# Autodesk Inventor assembly: 000-hand-grab-v5
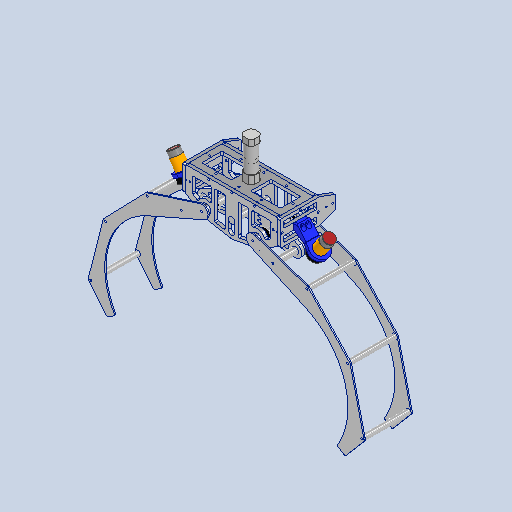
[picture p0: Inventor's stored thumbnail of the model, 512x512]
Saved by Autodesk Inventor 2025.2 (Build 292293000, 293)
## iProperties
Created: 2025-05-11
Part Number: 000-hand-grab-v5
Document SubType Name: Assembly
Designer: haruy
Author: haruy
## Documents named in this file (17)
- C:\Users\haruy\Documents\ロボコン\NHK2025\cad\nagahisa\hand\grab\000-hand-grab-v5.iam
- C:\Users\haruy\Documents\ロボコン\NHK2025\cad\nagahisa\hand\grab\hand-grab-v5-Plate-1.ipt
- C:\Users\haruy\Documents\ロボコン\NHK2025\cad\000_parts\エアシリンダー\airclinder\CDJ2B16-15Z-B(0_1_0).iam
- C:\Users\haruy\Documents\ロボコン\NHK2025\cad\nagahisa\hand\grab\hand-grab-v5-Plate-2.ipt
- C:\Users\haruy\Documents\ロボコン\NHK2025\cad\nagahisa\hand\grab\hand-grab-v5-Plate-3.ipt
- C:\Users\haruy\Documents\ロボコン\NHK2025\cad\000_parts\ベアリング\10\bear_10_15_sn.ipt
- C:\Users\haruy\Documents\ロボコン\NHK2025\cad\nagahisa\belt_liner\SCBRJ10-13.iam
- C:\Users\haruy\Documents\ロボコン\NHK2025\cad\nagahisa\hand\grab\hand-grab-v5-shaft-1.ipt
- C:\Users\haruy\Documents\ロボコン\NHK2025\cad\nagahisa\hand\grab\hand-grab-v5-Plate-4.ipt
- C:\Users\haruy\Documents\ロボコン\NHK2025\cad\nagahisa\hand\grab\hand-grab-v5-Plate-5.ipt
- C:\Users\haruy\Documents\ロボコン\NHK2025\cad\nagahisa\hand\grab\000-hand-grab-v5\デザイン アクセラレータ\平歯車1.iam
- C:\Users\haruy\Documents\ロボコン\NHK2025\cad\nagahisa\belt_liner\PSCTW10.iam
- C:\Users\haruy\Documents\ロボコン\NHK2025\cad\nagahisa\hand\grab\hand-grab-v5-shaft-2.ipt
- C:\Users\haruy\Documents\ロボコン\NHK2025\cad\nagahisa\hand\grab\hand-grab-v5-shaft-3.ipt
- C:\Users\haruy\Documents\ロボコン\NHK2025\cad\nagahisa\hand\grab\hand-grab-v5-3DP-1.ipt
- C:\Users\haruy\Documents\ロボコン\NHK2025\cad\000_parts\センサー\E18_D80NK.ipt
- C:\Users\haruy\Documents\ロボコン\NHK2025\cad\nagahisa\hand\grab\hand-grab-v5-shaft-4.ipt
## Components (38 placed, 16 different names)
1. hand-grab-v5-Plate-1:1 — 挿入:1, 角度:1, フラッシュ:7, メイト:3, メイト:4, フラッシュ:10, メイト:6, フラッシュ:12, メイト:8, フラッシュ:13
2. CDJ2B16-15Z-B(0_1_0):1 [sub-assembly] — 挿入:1, 挿入:2
3. hand-grab-v5-Plate-2:1 — 挿入:2, 角度:1, 挿入:27, フラッシュ:14
4. bear_10_15_sn:1 — 挿入:9, 挿入:22
5. bear_10_15_sn:2 — 挿入:10, 挿入:23
6. bear_10_15_sn:3 — 挿入:8, 挿入:21
7. bear_10_15_sn:4 — 挿入:7, 挿入:20
8. SCBRJ10-13:1 [sub-assembly] — 挿入:7, 挿入:46
9. SCBRJ10-13:2 [sub-assembly] — 挿入:8
10. SCBRJ10-13:3 [sub-assembly] — 挿入:9, 挿入:48
11. SCBRJ10-13:4 [sub-assembly] — 挿入:10
12. hand-grab-v5-shaft-1:1 — 挿入:15, 挿入:16, 挿入:25
13. hand-grab-v5-shaft-1:2 — 挿入:13, 挿入:14, 挿入:24
14. hand-grab-v5-Plate-4:1 — 挿入:13, 挿入:29, 挿入:32, 挿入:39, 挿入:51
15. hand-grab-v5-Plate-4:2 — 挿入:14, 挿入:28, 挿入:33, 挿入:38
16. hand-grab-v5-Plate-4:3 — 挿入:16, 挿入:30, 挿入:35, 挿入:37, 挿入:53
17. hand-grab-v5-Plate-4:4 — 挿入:15, 挿入:31, 挿入:34, 挿入:36
18. hand-grab-v5-Plate-5:1 — メイト:4, フラッシュ:10, メイト:7, 挿入:42, 挿入:43
19. hand-grab-v5-Plate-5:2 — フラッシュ:7, メイト:3, メイト:9, 挿入:40, 挿入:41
20. 平歯車:1 [sub-assembly] — 挿入:46, 挿入:47, 挿入:50
21. PSCTW10:1 [sub-assembly] — 挿入:47
22. 平歯車:2 [sub-assembly] — 挿入:48, 挿入:49, フラッシュ:14, 挿入:52
23. PSCTW10:2 [sub-assembly] — 挿入:49
24. hand-grab-v5-Plate-3:1 — メイト:6, フラッシュ:12, メイト:7, 挿入:20, 挿入:22, 挿入:24, 挿入:25
25. hand-grab-v5-Plate-3:2 — メイト:8, フラッシュ:13, メイト:9, 挿入:21, 挿入:23
26. hand-grab-v5-shaft-2:1 — 挿入:27
27. hand-grab-v5-shaft-3:1 — 挿入:28, 挿入:29
28. hand-grab-v5-shaft-3:2 — 挿入:30, 挿入:31
29. hand-grab-v5-shaft-3:3 — 挿入:32, 挿入:33
30. hand-grab-v5-shaft-3:4 — 挿入:34, 挿入:35
31. hand-grab-v5-shaft-3:5 — 挿入:36, 挿入:37
32. hand-grab-v5-shaft-3:6 — 挿入:38, 挿入:39
33. hand-grab-v5-3DP-1:1 — 挿入:40, 挿入:41, 挿入:44
34. hand-grab-v5-3DP-1:2 — 挿入:42, 挿入:43, 挿入:45
35. E18_D80NK:1 — 挿入:44
36. E18_D80NK:2 — 挿入:45
37. hand-grab-v5-shaft-4:1 — 挿入:50, 挿入:51
38. hand-grab-v5-shaft-4:2 — 挿入:52, 挿入:53
## Relationships (55: Insert 43, Mate 6, Flush 5, Angle 1)
- 挿入:1 [Insert]: hand-grab-v5-Plate-1:1 ↔ CDJ2B16-15Z-B(0_1_0):1
- 挿入:2 [Insert] (5.5 mm): CDJ2B16-15Z-B(0_1_0):1 ↔ hand-grab-v5-Plate-2:1
- 角度:1 [Angle] (0 deg): hand-grab-v5-Plate-1:1 ↔ hand-grab-v5-Plate-2:1
- 挿入:7 [Insert]: bear_10_15_sn:4 ↔ SCBRJ10-13:1
- 挿入:8 [Insert]: bear_10_15_sn:3 ↔ SCBRJ10-13:2
- 挿入:9 [Insert]: bear_10_15_sn:1 ↔ SCBRJ10-13:3
- 挿入:10 [Insert]: bear_10_15_sn:2 ↔ SCBRJ10-13:4
- 挿入:13 [Insert]: hand-grab-v5-shaft-1:2 ↔ hand-grab-v5-Plate-4:1
- 挿入:14 [Insert]: hand-grab-v5-shaft-1:2 ↔ hand-grab-v5-Plate-4:2
- 挿入:15 [Insert]: hand-grab-v5-shaft-1:1 ↔ hand-grab-v5-Plate-4:4
- 挿入:16 [Insert]: hand-grab-v5-shaft-1:1 ↔ hand-grab-v5-Plate-4:3
- フラッシュ:7 [Flush]: hand-grab-v5-Plate-1:1 ↔ hand-grab-v5-Plate-5:2
- メイト:3 [Mate]: hand-grab-v5-Plate-1:1 ↔ hand-grab-v5-Plate-5:2
- メイト:4 [Mate]: hand-grab-v5-Plate-1:1 ↔ hand-grab-v5-Plate-5:1
- フラッシュ:10 [Flush]: hand-grab-v5-Plate-1:1 ↔ hand-grab-v5-Plate-5:1
- メイト:6 [Mate]: hand-grab-v5-Plate-1:1 ↔ hand-grab-v5-Plate-3:1
- フラッシュ:12 [Flush]: hand-grab-v5-Plate-1:1 ↔ hand-grab-v5-Plate-3:1
- メイト:7 [Mate]: hand-grab-v5-Plate-5:1 ↔ hand-grab-v5-Plate-3:1
- メイト:8 [Mate]: hand-grab-v5-Plate-1:1 ↔ hand-grab-v5-Plate-3:2
- フラッシュ:13 [Flush]: hand-grab-v5-Plate-1:1 ↔ hand-grab-v5-Plate-3:2
- メイト:9 [Mate]: hand-grab-v5-Plate-5:2 ↔ hand-grab-v5-Plate-3:2
- 挿入:20 [Insert]: bear_10_15_sn:4 ↔ hand-grab-v5-Plate-3:1
- 挿入:21 [Insert]: bear_10_15_sn:3 ↔ hand-grab-v5-Plate-3:2
- 挿入:22 [Insert]: bear_10_15_sn:1 ↔ hand-grab-v5-Plate-3:1
- 挿入:23 [Insert]: bear_10_15_sn:2 ↔ hand-grab-v5-Plate-3:2
- 挿入:24 [Insert] (5 mm): hand-grab-v5-shaft-1:2 ↔ hand-grab-v5-Plate-3:1
- 挿入:25 [Insert] (5 mm): hand-grab-v5-shaft-1:1 ↔ hand-grab-v5-Plate-3:1
- 挿入:27 [Insert] (-28.5 mm): hand-grab-v5-Plate-2:1 ↔ hand-grab-v5-shaft-2:1
- 挿入:28 [Insert]: hand-grab-v5-Plate-4:2 ↔ hand-grab-v5-shaft-3:1
- 挿入:29 [Insert]: hand-grab-v5-Plate-4:1 ↔ hand-grab-v5-shaft-3:1
- 挿入:30 [Insert]: hand-grab-v5-Plate-4:3 ↔ hand-grab-v5-shaft-3:2
- 挿入:31 [Insert]: hand-grab-v5-Plate-4:4 ↔ hand-grab-v5-shaft-3:2
- 挿入:32 [Insert]: hand-grab-v5-Plate-4:1 ↔ hand-grab-v5-shaft-3:3
- 挿入:33 [Insert]: hand-grab-v5-Plate-4:2 ↔ hand-grab-v5-shaft-3:3
- 挿入:34 [Insert]: hand-grab-v5-Plate-4:4 ↔ hand-grab-v5-shaft-3:4
- 挿入:35 [Insert]: hand-grab-v5-Plate-4:3 ↔ hand-grab-v5-shaft-3:4
- 挿入:36 [Insert]: hand-grab-v5-Plate-4:4 ↔ hand-grab-v5-shaft-3:5
- 挿入:37 [Insert]: hand-grab-v5-Plate-4:3 ↔ hand-grab-v5-shaft-3:5
- 挿入:38 [Insert]: hand-grab-v5-Plate-4:2 ↔ hand-grab-v5-shaft-3:6
- 挿入:39 [Insert]: hand-grab-v5-Plate-4:1 ↔ hand-grab-v5-shaft-3:6
- 挿入:40 [Insert]: hand-grab-v5-Plate-5:2 ↔ hand-grab-v5-3DP-1:1
- 挿入:41 [Insert]: hand-grab-v5-Plate-5:2 ↔ hand-grab-v5-3DP-1:1
- 挿入:42 [Insert]: hand-grab-v5-Plate-5:1 ↔ hand-grab-v5-3DP-1:2
- 挿入:43 [Insert]: hand-grab-v5-Plate-5:1 ↔ hand-grab-v5-3DP-1:2
- 挿入:44 [Insert]: hand-grab-v5-3DP-1:1 ↔ E18_D80NK:1
- 挿入:45 [Insert]: hand-grab-v5-3DP-1:2 ↔ E18_D80NK:2
- 挿入:46 [Insert] (15 mm): SCBRJ10-13:1 ↔ 平歯車:1
- 挿入:47 [Insert]: 平歯車:1 ↔ PSCTW10:1
- 挿入:48 [Insert] (15 mm): SCBRJ10-13:3 ↔ 平歯車:2
- 挿入:49 [Insert]: 平歯車:2 ↔ PSCTW10:2
- フラッシュ:14 [Flush]: hand-grab-v5-Plate-2:1 ↔ 平歯車:2
- 挿入:50 [Insert] (-33.5 mm): 平歯車:1 ↔ hand-grab-v5-shaft-4:1
- 挿入:51 [Insert]: hand-grab-v5-Plate-4:1 ↔ hand-grab-v5-shaft-4:1
- 挿入:52 [Insert] (-33.5 mm): 平歯車:2 ↔ hand-grab-v5-shaft-4:2
- 挿入:53 [Insert]: hand-grab-v5-Plate-4:3 ↔ hand-grab-v5-shaft-4:2
